# Autodesk Inventor assembly: tibia kanan
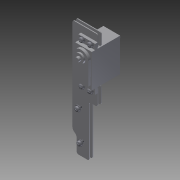
[picture p0: Inventor's stored thumbnail of the model, 180x180]
Saved by Autodesk Inventor 2012 (Build 160160000, 160)
## iProperties
Created: 2013-12-05
Part Number: tibia kanan
Document SubType Name: Assembly
Designer: Irwan Haryanto
Author: Irwan Haryanto
## Documents named in this file (4)
- D:\Revenant\robot baru 2014\tibia kanan.iam
- D:\Revenant\robot baru 2014\riset tibia alumunium 1.ipt
- D:\Revenant\robot baru 2014\servo HS-7955GT.ipt
- D:\Revenant\robot baru 2014\tibia kanan\Design Accelerator\Bolted Connection1.iam
## Components (4 placed, 3 different names)
1. riset tibia alumunium 1:1 — Insert:1, Insert:2, Insert:3, Insert:4, Insert:5, Insert:6
2. riset tibia alumunium 1:2 — Insert:5, Insert:6, Mate:2
3. servo HS-7955GT:1 — Insert:1, Insert:2, Insert:3, Insert:4, Mate:1
4. Bolted Connection:1 [sub-assembly] — Mate:1, Mate:2
## Relationships (8: Insert 6, Mate 2)
- Insert:1: riset tibia alumunium 1:1 ↔ servo HS-7955GT:1
- Insert:2: riset tibia alumunium 1:1 ↔ servo HS-7955GT:1
- Insert:3: riset tibia alumunium 1:1 ↔ servo HS-7955GT:1
- Insert:4: riset tibia alumunium 1:1 ↔ servo HS-7955GT:1
- Insert:5 (3 mm): riset tibia alumunium 1:1 ↔ riset tibia alumunium 1:2
- Insert:6: riset tibia alumunium 1:1 ↔ riset tibia alumunium 1:2
- Mate:1: servo HS-7955GT:1 ↔ Bolted Connection:1
- Mate:2: riset tibia alumunium 1:2 ↔ Bolted Connection:1
